# Autodesk Inventor assembly: ASDSAssembly
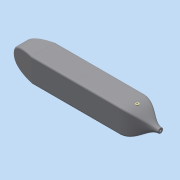
[picture p0: Inventor's stored thumbnail of the model, 180x180]
Saved by Autodesk Inventor 2017 (Build 210142000, 142)
## iProperties
Created: 2017-02-12
Part Number: ASDSAssembly
Document SubType Name: Assembly
Designer: techn
Author: techn
## Documents named in this file (6)
- D:\OneDrive\Documents\Other Projects\Submarine\CAD\ASDS\ASDSAssembly.iam
- D:\OneDrive\Documents\Other Projects\Submarine\CAD\ASDS\Fore.ipt
- D:\OneDrive\Documents\Other Projects\Submarine\CAD\ASDS\MidshipsHullFrontSection.ipt
- D:\OneDrive\Documents\Other Projects\Submarine\CAD\ASDS\MidshipsHullRearSection.ipt
- D:\OneDrive\Documents\Other Projects\Submarine\CAD\ASDS\Aft.ipt
- D:\OneDrive\Documents\Other Projects\Submarine\CAD\ASDS\shoulderWasher.ipt
## Components (6 placed, 5 different names)
1. Fore:1 — Mate:1, Mate:2, Mate:3
2. MidshipsHullFrontSection:1 — Mate:1, Mate:2, Mate:3, Mate:4, Mate:5, Mate:6
3. MidshipsHullRearSection:1 — Mate:4, Mate:5, Mate:6, Mate:7, Mate:8, Mate:9
4. Aft:1 — Mate:7, Mate:8, Mate:9, Mate:10, Mate:11, Mate:12, Mate:13
5. shoulderWasher:1 — Mate:10, Mate:13
6. shoulderWasher:2 — Mate:11, Mate:12
## Relationships (13: Mate 13)
- Mate:1: Fore:1 ↔ MidshipsHullFrontSection:1
- Mate:2: Fore:1 ↔ MidshipsHullFrontSection:1
- Mate:3: Fore:1 ↔ MidshipsHullFrontSection:1
- Mate:4: MidshipsHullFrontSection:1 ↔ MidshipsHullRearSection:1
- Mate:5: MidshipsHullFrontSection:1 ↔ MidshipsHullRearSection:1
- Mate:6: MidshipsHullFrontSection:1 ↔ MidshipsHullRearSection:1
- Mate:7: MidshipsHullRearSection:1 ↔ Aft:1
- Mate:8: MidshipsHullRearSection:1 ↔ Aft:1
- Mate:9: MidshipsHullRearSection:1 ↔ Aft:1
- Mate:10: Aft:1 ↔ shoulderWasher:1
- Mate:11: Aft:1 ↔ shoulderWasher:2
- Mate:12: Aft:1 ↔ shoulderWasher:2
- Mate:13: Aft:1 ↔ shoulderWasher:1
